# Autodesk Inventor assembly: Q5_Fan_Assem
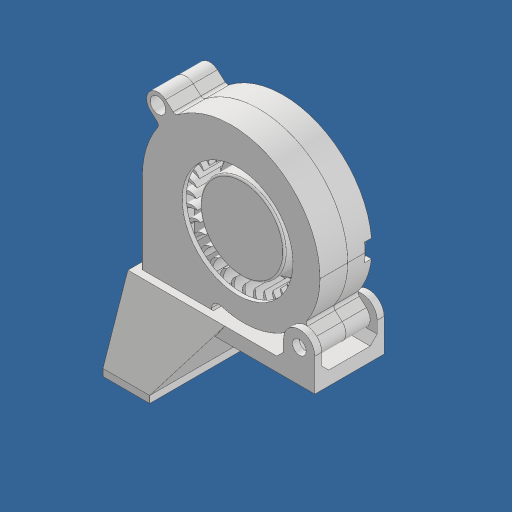
[picture p0: Inventor's stored thumbnail of the model, 512x512]
Saved by Autodesk Inventor 2024.2 (Build 282272000, 272)
## iProperties
Created: 2024-06-06
Part Number: Q5_Fan_Assem
Document SubType Name: Assembly
Designer: Charlie Kendall
Author: Charlie Kendall
## Documents named in this file (3)
- E:\1char\Documents\Q5\Q5_Fan_Assem.iam
- E:\1char\Documents\Q5\Fan_Duct_1.ipt
- E:\1char\Documents\Q5\Fan 5015\Fan 5015.ipt
## Components (2 placed, 2 different names)
1. Fan_Duct_1:1 — Mate:1, Mate:2, Mate:3
2. Fan 5015:1 — Mate:1, Mate:2, Mate:3
## Relationships (3: Mate 3)
- Mate:1: Fan_Duct_1:1 ↔ Fan 5015:1
- Mate:2: Fan_Duct_1:1 ↔ Fan 5015:1
- Mate:3: Fan_Duct_1:1 ↔ Fan 5015:1
